# Autodesk Inventor assembly: Drawer Assembly
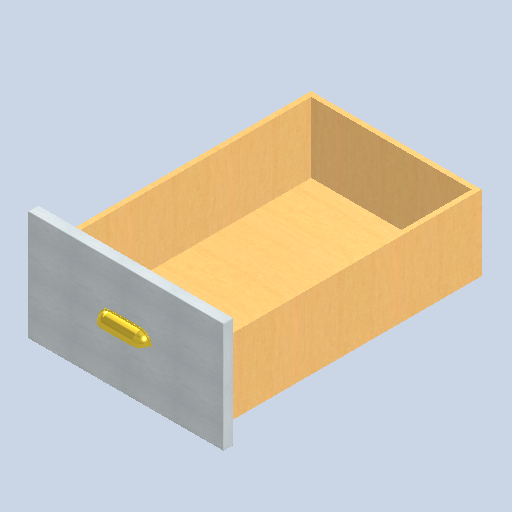
[picture p0: Inventor's stored thumbnail of the model, 512x512]
Saved by Autodesk Inventor 2022 (Build 260153000, 153)
## iProperties
Company: Jay's Dressers
RuleStatus: InUse
Created: 2021-10-04
Document SubType Name: Assembly
Designer: Admin
Author: Admin
Title: Drawer Assembly
## Documents named in this file (6)
- C:\Users\Admin\source\repos\DresserWebApplication\DresserAutomationPlugin\Resources\Dresser Base Model\Drawer\Drawer Assembly.iam
- C:\Users\Admin\source\repos\DresserWebApplication\DresserAutomationPlugin\Resources\Dresser Base Model\Drawer\Drawer Bottom.ipt
- C:\Users\Admin\source\repos\DresserWebApplication\DresserAutomationPlugin\Resources\Dresser Base Model\Drawer\Drawer Front Panel.ipt
- C:\Users\Admin\source\repos\DresserWebApplication\DresserAutomationPlugin\Resources\Dresser Base Model\Drawer\Drawer Side Panel.ipt
- C:\Users\Admin\source\repos\DresserWebApplication\DresserAutomationPlugin\Resources\Dresser Base Model\Drawer\Drawer Back Panel.ipt
- C:\Users\Admin\source\repos\DresserWebApplication\DresserAutomationPlugin\Resources\Dresser Base Model\Drawer\Hardware\Bin Pull.ipt
## Components (6 placed, 5 different names)
1. Drawer Bottom:1 — Mate:1, Flush:1, Mate:2, Mate:4, Flush:3, Flush:4, Mate:6, Flush:5
2. Drawer Front Panel:1 — Mate:1, Flush:1, Flush:2, Mate:3, Mate:5
3. Drawer Side Panel:1 — Mate:2, Mate:3, Flush:3
4. Drawer Side Panel:2 — Mate:4, Mate:5, Flush:4
5. Drawer Back Panel:1 — Mate:6, Flush:5, Flush:6
6. Handle
## Relationships (15: Flush 8, Mate 7)
- Mate:1: Drawer Bottom:1 ↔ Drawer Front Panel:1
- Flush:1 (-25.4 mm): Drawer Bottom:1 ↔ Drawer Front Panel:1
- Flush:2: Drawer Front Panel:1
- Mate:2: Drawer Bottom:1 ↔ Drawer Side Panel:1
- Mate:3: Drawer Front Panel:1 ↔ Drawer Side Panel:1
- Mate:4: Drawer Bottom:1 ↔ Drawer Side Panel:2
- Mate:5: Drawer Front Panel:1 ↔ Drawer Side Panel:2
- Flush:3: Drawer Bottom:1 ↔ Drawer Side Panel:1
- Flush:4: Drawer Bottom:1 ↔ Drawer Side Panel:2
- Mate:6: Drawer Bottom:1 ↔ Drawer Back Panel:1
- Flush:5: Drawer Bottom:1 ↔ Drawer Back Panel:1
- Flush:6: Drawer Back Panel:1
- [Flush]: Handle
- [Flush]: Drawer Front Panel:1 ↔ Handle
- [Mate]: Drawer Front Panel:1 ↔ Handle
